# Autodesk Inventor assembly: Y-Motor-Housing
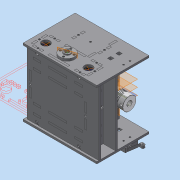
[picture p0: Inventor's stored thumbnail of the model, 180x180]
Saved by Autodesk Inventor 2016 SP1 (Build 200210100, 210)
## iProperties
Created: 2016-03-01
Part Number: Y-Motor-Housing
Document SubType Name: Assembly
Designer: Mohamed A.
Author: Mohamed A.
## Documents named in this file (14)
- C:\Users\Mohamed\Documents\inventor\Faboscope\Laser Cut\Y-Motor-Housing\new\Y-Motor-Housing.iam
- C:\Users\Mohamed\Documents\inventor\Faboscope\Laser Cut\Y-Motor-Housing\new\Side.ipt
- C:\Users\Mohamed\Documents\inventor\Faboscope\Lead Screws\8mm flanged lead screw nut with 2mm thread.ipt
- C:\Users\Mohamed\Documents\inventor\Faboscope\Motors\NEMA-7-17HD34008-22B.ipt
- C:\Users\Mohamed\Documents\inventor\Faboscope\Bearings\LM8UU 8mm Linear Bearing.ipt
- C:\Users\Mohamed\Documents\inventor\Faboscope\Couplers\Flexible Shaft CouplerAcople FlexibleSLDPRT.ipt
- C:\Users\Mohamed\Documents\inventor\Faboscope\Buttons\SPDT Limit Switch\605634.ipt
- C:\Users\Mohamed\Documents\inventor\Faboscope\Laser Cut\Y-Motor-Housing\new\Front-Inner.ipt
- C:\Users\Mohamed\Documents\inventor\Faboscope\Laser Cut\Y-Motor-Housing\new\Base.ipt
- C:\Users\Mohamed\Documents\inventor\Faboscope\Laser Cut\Y-Motor-Housing\new\Bearing-Outer.ipt
- C:\Users\Mohamed\Documents\inventor\Faboscope\Laser Cut\Y-Motor-Housing\new\Bearing-Middle.ipt
- C:\Users\Mohamed\Documents\inventor\Faboscope\Laser Cut\Y-Motor-Housing\new\Bearing-Side.ipt
- C:\Users\Mohamed\Documents\inventor\Faboscope\Laser Cut\Y-Motor-Housing\new\Bearing-Bottom.ipt
- C:\Users\Mohamed\Documents\inventor\Faboscope\Laser Cut\Y-Motor-Housing\new\Front-Outer.ipt
## Components (21 placed, 13 different names)
1. Side:1 — Flush:5
2. 8mm flanged lead screw nut with 2mm thread:1 — Mate:4, Mate:5
3. NEMA-7-17HD34008-22B:1 — Mate:3, Flush:6
4. LM8UU 8mm Linear Bearing:1
5. LM8UU 8mm Linear Bearing:2 — Mate:1
6. Flexible Shaft CouplerAcople FlexibleSLDPRT:1
7. 605634:1
8. Front-Inner:1
9. Base:1 — Flush:1, Flush:4
10. Bearing-Outer:1 — Mate:1, Flush:1, Flush:2
11. Bearing-Middle:1
12. Bearing-Side:1 — Flush:2, Flush:3
13. Bearing-Side:2
14. Side:2 — Mate:4, Mate:5
15. LM8UU 8mm Linear Bearing:3 — Mate:2
16. LM8UU 8mm Linear Bearing:4
17. Bearing-Middle:2
18. Bearing-Outer:2 — Mate:2, Flush:3, Flush:4
19. Bearing-Bottom:1
20. Front-Outer:1
21. Front-Outer:2 — Mate:3, Flush:5, Flush:6
## Relationships (11: Flush 6, Mate 5)
- Mate:1: LM8UU 8mm Linear Bearing:2 ↔ Bearing-Outer:1
- Flush:1: Base:1 ↔ Bearing-Outer:1
- Flush:2: Bearing-Outer:1 ↔ Bearing-Side:1
- Mate:2: LM8UU 8mm Linear Bearing:3 ↔ Bearing-Outer:2
- Flush:3: Bearing-Side:1 ↔ Bearing-Outer:2
- Flush:4: Base:1 ↔ Bearing-Outer:2
- Mate:3: NEMA-7-17HD34008-22B:1 ↔ Front-Outer:2
- Flush:5: Side:1 ↔ Front-Outer:2
- Flush:6: NEMA-7-17HD34008-22B:1 ↔ Front-Outer:2
- Mate:4: 8mm flanged lead screw nut with 2mm thread:1 ↔ Side:2
- Mate:5: 8mm flanged lead screw nut with 2mm thread:1 ↔ Side:2
